# Autodesk Inventor assembly: Baugruppe1
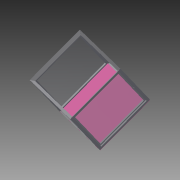
[picture p0: Inventor's stored thumbnail of the model, 180x180]
Saved by Autodesk Inventor 2018.2 (Build 222227000, 227)
## iProperties
Created: 2019-09-20
Part Number: Baugruppe1
Material: Generisch
Document SubType Name: Assembly
Designer: Lolob
Author: Lolob
## Documents named in this file (10)
- C:\Users\Lolob\Documents\Dipl\Smartcube_Construction\Version_3\Baugruppe1.iam
- C:\Users\Lolob\Documents\Dipl\Smartcube_Construction\Version_2\PV_Ramen.ipt
- C:\Users\Lolob\Documents\Dipl\Smartcube_Construction\Version_2\PV_Modul.ipt
- C:\Users\Lolob\Documents\Dipl\Smartcube_Construction\Version_2\PV_Ramen_CPY.ipt
- C:\Users\Lolob\Documents\Dipl\Smartcube_Construction\Version_2\PV_Modul_CPY.ipt
- C:\Users\Lolob\Documents\Dipl\Smartcube_Construction\Version_2\PV_Ramen_CPY_3.ipt
- C:\Users\Lolob\Documents\Dipl\Smartcube_Construction\Version_2\PV_Modul_CPY_3.ipt
- C:\Users\Lolob\Documents\Dipl\Smartcube_Construction\Version_2\PV_Ramen_CPY_3_3.ipt
- C:\Users\Lolob\Documents\Dipl\Smartcube_Construction\Version_2\PV_Modul_CPY_3_3.ipt
- C:\Users\Lolob\Documents\Dipl\Smartcube_Construction\Version_3\Boden.ipt
## Components (9 placed, 9 different names)
1. PV_Ramen:1 — Starr:1, Starr:3, Passend:2, Passend:3
2. PV_Modul:1 — Starr:1
3. PV_Ramen_CPY:1 — Starr:2, Starr:3, Starr:5
4. PV_Modul_CPY:1 — Starr:2
5. PV_Ramen_CPY_3:1 — Starr:4, Starr:5, Starr:7
6. PV_Modul_CPY_3:1 — Starr:4
7. PV_Ramen_CPY_3_3:1 — Starr:6, Starr:7, Passend:1, Starr:8
8. PV_Modul_CPY_3_3:1 — Starr:6
9. Boden:1 — Starr:8
## Relationships (11: WeldJoint 8, Mate 3)
- Starr:1 [WeldJoint]: PV_Ramen:1 ↔ PV_Modul:1
- Starr:2 [WeldJoint]: PV_Ramen_CPY:1 ↔ PV_Modul_CPY:1
- Starr:3 [WeldJoint]: PV_Ramen:1 ↔ PV_Ramen_CPY:1
- Starr:4 [WeldJoint]: PV_Ramen_CPY_3:1 ↔ PV_Modul_CPY_3:1
- Starr:5 [WeldJoint]: PV_Ramen_CPY:1 ↔ PV_Ramen_CPY_3:1
- Starr:6 [WeldJoint]: PV_Ramen_CPY_3_3:1 ↔ PV_Modul_CPY_3_3:1
- Starr:7 [WeldJoint]: PV_Ramen_CPY_3:1 ↔ PV_Ramen_CPY_3_3:1
- Passend:1 [Mate]: PV_Ramen_CPY_3_3:1
- Passend:2 [Mate]: PV_Ramen:1
- Passend:3 [Mate]: PV_Ramen:1
- Starr:8 [WeldJoint]: PV_Ramen_CPY_3_3:1 ↔ Boden:1
